# Autodesk Inventor assembly: Antriebsstrang
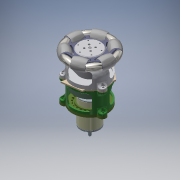
[picture p0: Inventor's stored thumbnail of the model, 180x180]
Saved by Autodesk Inventor 2018.3 (Build 223284000, 284)
## iProperties
Created: 2018-06-25
Part Number: Antriebsstrang
Material: Generisch
Document SubType Name: Assembly
Designer: JochenAlt
Author: JochenAlt
## Documents named in this file (6)
- D:\Projects\FlowerPot\CAD\DriveChain.iam
- D:\Projects\FlowerPot\CAD\OmniWheel.ipt
- D:\Projects\FlowerPot\CAD\HarmonicDrive.iam
- D:\Projects\FlowerPot\CAD\Mounting Hub.ipt
- C:\Users\JochenAlt\Documents\Inventor\Content Center Files\R2018\de-DE\SKF - Single row ball bearings\SKF604.ipt
- D:\Projects\FlowerPot\CAD\Avago Encoder.iam
## Components (5 placed, 5 different names)
1. OmniWheel:1 — Passend:6, Passend:7, Passend:8
2. HarmonicDrive:1 [sub-assembly] — Passend:4, Passend:5, Passend:6, Passend:9, Passend:10, Passend:11, Passend:13, Winkel:1
3. Mounting Hub:1 — Passend:5, Passend:7, Passend:8, Passend:10
4. SKF- Kugellager, einreihig SKF604:1 — Passend:4, Passend:9
5. Avago Encoder:1 [sub-assembly] — Passend:11, Passend:13, Winkel:1
## Relationships (10: Mate 9, Angle 1)
- Passend:4 [Mate]: HarmonicDrive:1 ↔ SKF- Kugellager, einreihig SKF604:1
- Passend:5 [Mate]: HarmonicDrive:1 ↔ Mounting Hub:1
- Passend:6 [Mate]: OmniWheel:1 ↔ HarmonicDrive:1
- Passend:7 [Mate]: OmniWheel:1 ↔ Mounting Hub:1
- Passend:8 [Mate]: OmniWheel:1 ↔ Mounting Hub:1
- Passend:9 [Mate]: HarmonicDrive:1 ↔ SKF- Kugellager, einreihig SKF604:1
- Passend:10 [Mate] (1 mm): HarmonicDrive:1 ↔ Mounting Hub:1
- Passend:11 [Mate]: HarmonicDrive:1 ↔ Avago Encoder:1
- Passend:13 [Mate] (0.5 mm): HarmonicDrive:1 ↔ Avago Encoder:1
- Winkel:1 [Angle] (180 deg): HarmonicDrive:1 ↔ Avago Encoder:1
